# Autodesk Inventor assembly: 42 t pulley
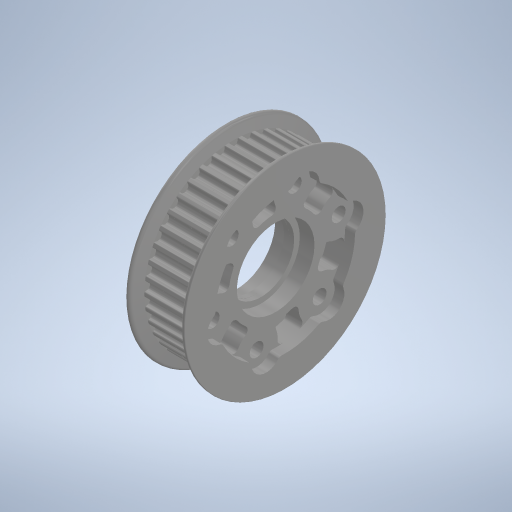
[picture p0: Inventor's stored thumbnail of the model, 512x512]
Saved by Autodesk Inventor 2023 (Build 270158000, 158)
## iProperties
Created: 2023-03-29
Part Number: 42 t pulley
Document SubType Name: Assembly
Designer: Gabriel - T3 CAD
Author: Gabriel - T3 CAD
## Documents named in this file (2)
- C:\Users\Gabriel - T3 CAD\Documents\GitHub\T3-CAD\Stock\Belts-Chain\Belts\HTD\15 mm Width\42 t pulley.iam
- C:\Users\Gabriel - T3 CAD\Documents\GitHub\T3-CAD\Stock\Belts-Chain\Belts\HTD\15 mm Width\am-2234a_half 42 tooth HTD Pulley half.ipt
## Components (2 placed, 1 different names)
1. am-2234a_half 42 tooth HTD Pulley half:1 — Rotational:1, Rotational:2
2. am-2234a_half 42 tooth HTD Pulley half:2 — Rotational:1, Rotational:2
## Relationships (2: RevoluteJoint 2)
- Rotational:1 [RevoluteJoint]: am-2234a_half 42 tooth HTD Pulley half:1 ↔ am-2234a_half 42 tooth HTD Pulley half:2
- Rotational:2 [RevoluteJoint]: am-2234a_half 42 tooth HTD Pulley half:1 ↔ am-2234a_half 42 tooth HTD Pulley half:2
